# Autodesk Inventor assembly: bibrake
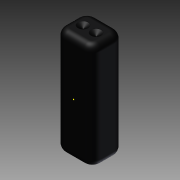
[picture p0: Inventor's stored thumbnail of the model, 180x180]
Saved by Autodesk Inventor 2017 (Build 210142000, 142)
## iProperties
Created: 2018-09-03
Part Number: bibrake
Document SubType Name: Assembly
Designer: ari
Author: ari
## Documents named in this file (3)
- C:\Users\ari\Documents\Inventor\bibrake\bibrake.iam
- C:\Users\ari\Documents\Inventor\bibrake\wire clamp egg.ipt
- C:\Users\ari\Documents\Inventor\bibrake\cable case standoff.ipt
## Components (2 placed, 2 different names)
1. wire clamp egg:1 — Mate:1
2. cable case standoff:1 — Mate:1
## Relationships (1: Mate 1)
- Mate:1 (3.5 mm): wire clamp egg:1 ↔ cable case standoff:1
